# Autodesk Inventor assembly: ARMV2
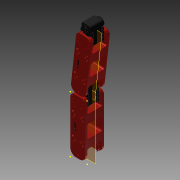
[picture p0: Inventor's stored thumbnail of the model, 180x180]
Saved by Autodesk Inventor 2015 (Build 190159000, 159)
## iProperties
Created: 2016-12-08
Part Number: ARMV2
Document SubType Name: Assembly
Designer: Rudge-Top
Author: Rudge-Top
## Documents named in this file (4)
- C:\Users\Rudge-Top\Documents\RoboticArm\Inventor 2015\ARMV2.iam
- C:\Users\Rudge-Top\Documents\RoboticArm\Inventor 2015\150mm Link_V2 PART A.ipt
- C:\Users\Rudge-Top\Documents\RoboticArm\Inventor 2015\150mm Link_V2 PART B.ipt
- C:\Users\Rudge-Top\Documents\RoboticArm\Inventor 2015\AX12.iam
## Components (6 placed, 3 different names)
1. 150mm Link_V2 PART A:1 — Insert:5, Flush:2
2. 150mm Link_V2 PART B:1 — Mate:3, Insert:4, Insert:5, Flush:2
3. AX12:1 [sub-assembly] — Mate:2, Insert:3, Mate:3, Insert:4
4. 150mm Link_V2 PART A:2 — Insert:2, Flush:1
5. 150mm Link_V2 PART B:2 — Mate:1, Insert:1, Insert:2, Flush:1, Mate:2, Insert:3
6. AX12:2 [sub-assembly] — Mate:1, Insert:1
## Relationships (10: Insert 5, Mate 3, Flush 2)
- Mate:1: 150mm Link_V2 PART B:2 ↔ AX12:2
- Insert:1: 150mm Link_V2 PART B:2 ↔ AX12:2
- Insert:2: 150mm Link_V2 PART A:2 ↔ 150mm Link_V2 PART B:2
- Flush:1: 150mm Link_V2 PART A:2 ↔ 150mm Link_V2 PART B:2
- Mate:2: AX12:1 ↔ 150mm Link_V2 PART B:2
- Insert:3: AX12:1 ↔ 150mm Link_V2 PART B:2
- Mate:3: 150mm Link_V2 PART B:1 ↔ AX12:1
- Insert:4: 150mm Link_V2 PART B:1 ↔ AX12:1
- Insert:5: 150mm Link_V2 PART A:1 ↔ 150mm Link_V2 PART B:1
- Flush:2: 150mm Link_V2 PART A:1 ↔ 150mm Link_V2 PART B:1
